# Autodesk Inventor assembly: assembled
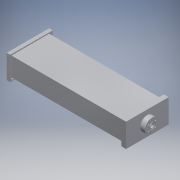
[picture p0: Inventor's stored thumbnail of the model, 180x180]
Saved by Autodesk Inventor 2016 (Build 200138000, 138)
## iProperties
Created: 2016-07-15
Part Number: assembled
Document SubType Name: Assembly
Designer: Jonathan
Author: Jonathan
## Documents named in this file (5)
- C:\Users\Jonathan\Desktop\Models\NuMu sensor\assembled.iam
- C:\Users\Jonathan\Desktop\Models\NuMu sensor\plateEnd.ipt
- C:\Users\Jonathan\Desktop\Models\NuMu sensor\tube.ipt
- C:\Users\Jonathan\Desktop\Models\NuMu sensor\0.375 in hole plate.ipt
- C:\Users\Jonathan\Desktop\Models\NuMu sensor\0.25 in hole.ipt
## Components (4 placed, 4 different names)
1. plateEnd:1 — Mate:4, Mate:5, Mate:7
2. tube:1 — Mate:4, Mate:5, Mate:6, Mate:7, Mate:9, Flush:1, Mate:10, Flush:2
3. 0.375 in hole plate:1 — Mate:6, Mate:8, Mate:9, Flush:1
4. 0.25 in hole:1 — Mate:8, Mate:10, Flush:2
## Relationships (9: Mate 7, Flush 2)
- Mate:4: plateEnd:1 ↔ tube:1
- Mate:5: plateEnd:1 ↔ tube:1
- Mate:6: tube:1 ↔ 0.375 in hole plate:1
- Mate:7: plateEnd:1 ↔ tube:1
- Mate:8: 0.375 in hole plate:1 ↔ 0.25 in hole:1
- Mate:9: tube:1 ↔ 0.375 in hole plate:1
- Flush:1: tube:1 ↔ 0.375 in hole plate:1
- Mate:10: tube:1 ↔ 0.25 in hole:1
- Flush:2: tube:1 ↔ 0.25 in hole:1
